# Autodesk Inventor assembly: Assembly1
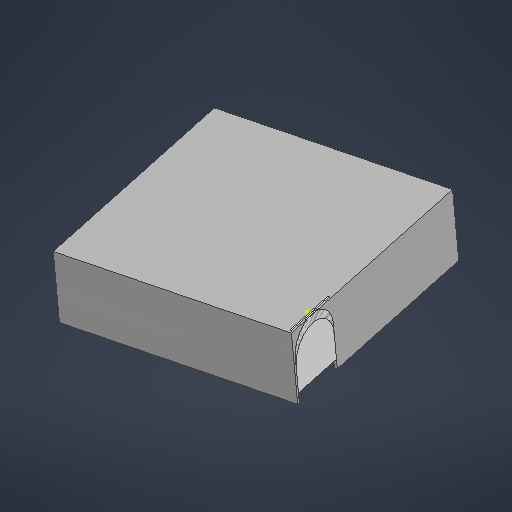
[picture p0: Inventor's stored thumbnail of the model, 512x512]
Saved by Autodesk Inventor 2026.1 (Build 301233000, 233)
## iProperties
Created: 2025-08-19
Part Number: Assembly1
Document SubType Name: Assembly
Designer: Paweł
Author: Paweł
## Documents named in this file (14)
- C:\Users\Paweł\OneDrive - Politechnika Warszawska\Dokumenty\gpstracker\Assembly1.iam
- C:\Users\Paweł\Downloads\esp-32-1.snapshot.6\ESP-32_v1\ESP-32_v1\ESP-32_v1.iam
- C:\Users\Paweł\Downloads\generic-li-ion-18650-cell-1.snapshot.4\Generic Li Ion 1850 cell\Generic Li Ion 1850 cell\18650_cell v1.ipt
- C:\Users\Paweł\Downloads\gy-neo6mv2-2.snapshot.2\GY-NEO6MV2-withAnt v7\GY-NEO6MV2-withAnt v7\GPS_ublox_board.iam
- C:\Users\Paweł\Downloads\gy-neo6mv2-2.snapshot.2\GY-NEO6MV2-withAnt v7\GY-NEO6MV2-withAnt v7\A_GPS_ant v2.iam
- C:\Users\Paweł\Downloads\mpu6050-8.snapshot.1\MPU6050 v2\MPU6050 v2\MPU6050 v2.ipt
- C:\Users\Paweł\Downloads\injoinic-ip2368-100w-usb-c-biderectional-powerbank-charging-board-module-1.snapshot.2\ip2368 v5\ip2368 v5\ip2368 v5.ipt
- C:\Users\Paweł\Downloads\sd-card-reader-4.snapshot.4\MicroSD Card Module - 1\MicroSD Card Module - 1\MicroSD Card Module - 1.iam
- C:\Users\Paweł\Downloads\micro-sd-card--1.snapshot.2\MicroSD.ipt
- C:\Users\Paweł\OneDrive - Politechnika Warszawska\Dokumenty\obudowa.ipt
- C:\Users\Paweł\Downloads\0-96-inch-oled-lcd-module-4-pin-128x64-1.snapshot.2\OSSD-128x64\OSSD-128x64\OSSD-128x64.ipt
- C:\Users\Paweł\Downloads\switch 15E20\switch 15E20\switch 15E20.ipt
- C:\Users\Paweł\OneDrive - Politechnika Warszawska\Dokumenty\gpstracker\pokrywka2.ipt
- C:\Users\Paweł\OneDrive - Politechnika Warszawska\Dokumenty\gpstracker\klapka.ipt
## Components (13 placed, 13 different names)
1. ESP-32_v1:1 [sub-assembly] — Mate:5
2. 18650_cell v1:1 — Insert:1, Insert:2
3. GPS_ublox_board:1 [sub-assembly] — Mate:13, Mate:15
4. A_GPS_ant v2:1 [sub-assembly] — Mate:21, Mate:22
5. MPU6050 v2:1 — Mate:7
6. ip2368 v5:1 — Mate:4
7. MicroSD Card Module - 1:1 [sub-assembly] — Mate:1, Mate:2, Mate:3, Mate:6
8. MicroSD:1 — Mate:1, Mate:2, Mate:3
9. obudowa:1 — Mate:4, Mate:5, Mate:6, Mate:7, Mate:10, Mate:13, Mate:14, Insert:1, Mate:23, Mate:24, Insert:2, Flush:1, Mate:25
10. OSSD-128x64:1 — Mate:17, Mate:18
11. switch 15E20:1 — Mate:10, Mate:14, Mate:15
12. pokrywka2:1 — Mate:17, Mate:18, Mate:21, Mate:22, Mate:23, Mate:24
13. klapka:1 — Flush:1, Mate:25
## Relationships (21: Mate 18, Insert 2, Flush 1)
- Mate:1: MicroSD Card Module - 1:1 ↔ MicroSD:1
- Mate:2: MicroSD Card Module - 1:1 ↔ MicroSD:1
- Mate:3: MicroSD Card Module - 1:1 ↔ MicroSD:1
- Mate:4: ip2368 v5:1 ↔ obudowa:1
- Mate:5: ESP-32_v1:1 ↔ obudowa:1
- Mate:6: MicroSD Card Module - 1:1 ↔ obudowa:1
- Mate:7: MPU6050 v2:1 ↔ obudowa:1
- Mate:10: obudowa:1 ↔ switch 15E20:1
- Mate:13: GPS_ublox_board:1 ↔ obudowa:1
- Mate:14: obudowa:1 ↔ switch 15E20:1
- Mate:15 (1 mm): GPS_ublox_board:1 ↔ switch 15E20:1
- Insert:1 (3 mm): 18650_cell v1:1 ↔ obudowa:1
- Mate:17: OSSD-128x64:1 ↔ pokrywka2:1
- Mate:18: OSSD-128x64:1 ↔ pokrywka2:1
- Mate:21: A_GPS_ant v2:1 ↔ pokrywka2:1
- Mate:22: A_GPS_ant v2:1 ↔ pokrywka2:1
- Mate:23: obudowa:1 ↔ pokrywka2:1
- Mate:24: obudowa:1 ↔ pokrywka2:1
- Insert:2 (2 mm): 18650_cell v1:1 ↔ obudowa:1
- Flush:1: obudowa:1 ↔ klapka:1
- Mate:25: obudowa:1 ↔ klapka:1
